# Autodesk Inventor assembly: joint3_frame
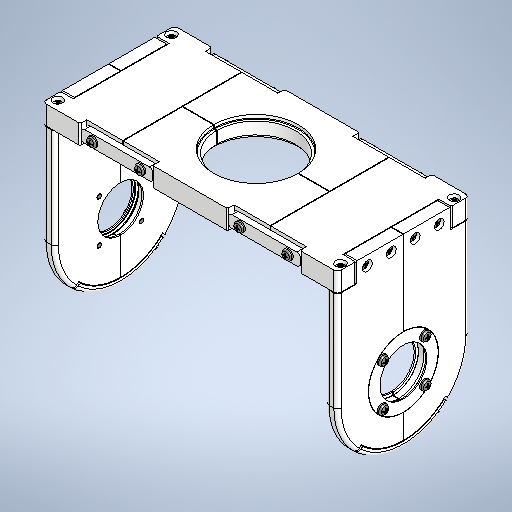
[picture p0: Inventor's stored thumbnail of the model, 512x512]
Saved by Autodesk Inventor 2025.3 (Build 293356030, 356C)
## iProperties
Created: 2025-11-25
Part Number: joint3_frame
Document SubType Name: Assembly
Designer: MSI
Mass: 762.261 g
Surface Area: 1764.87 cm^2
Volume: 601.306 cm^3
Density: 1.26767 g/cm^3
Author: MSI
## Documents named in this file (20)
- C:\Users\MSI\Desktop\Project\3. 로봇팔\Robot Arm Model\joint3\joint3_frame.iam
- C:\Users\MSI\Desktop\Project\3. 로봇팔\Robot Arm Model\joint3\joint3_frame_support1.ipt
- C:\Users\MSI\Desktop\Project\3. 로봇팔\Robot Arm Model\joint3\joint3_frame_support2.ipt
- C:\Users\MSI\Desktop\Project\3. 로봇팔\Robot Arm Model\joint3\joint3_frame1.ipt
- C:\Users\MSI\Desktop\Project\3. 로봇팔\Robot Arm Model\joint3\joint3_frame2.ipt
- C:\Users\MSI\Desktop\Project\3. 로봇팔\Robot Arm Model\joint3\carbon.ipt
- C:\Users\MSI\Desktop\Project\3. 로봇팔\Robot Arm Model\joint3\fixture.ipt
- C:\Users\MSI\Desktop\Project\3. 로봇팔\Robot Arm Model\joint3\joint3_frame_support_fixture.ipt
- C:\Users\MSI\Documents\Inventor\Content Center Files\R2025\ko-KR\KS B 1023  H (2)\KS B 1023 - A  M 4 x 16 - H(1).ipt
- C:\Users\MSI\Desktop\Project\3. 로봇팔\Robot Arm Model\joint3\fixture_MIR2.ipt
- C:\Users\MSI\Desktop\Project\3. 로봇팔\Robot Arm Model\joint3\joint3_frame_cover.ipt
- C:\Users\MSI\Documents\Inventor\Content Center Files\R2025\ko-KR\KS B 1023  H (2)\KS B 1023 - A  M 4 x 10 - H(1).ipt
- C:\Users\MSI\Desktop\Project\3. 로봇팔\Robot Arm Model\joint3\joint3_frame1_MIR.ipt
- C:\Users\MSI\Desktop\Project\3. 로봇팔\Robot Arm Model\joint3\fixture_MIR3.ipt
- C:\Users\MSI\Desktop\Project\3. 로봇팔\Robot Arm Model\joint3\fixture_MIR2_MIR.ipt
- C:\Users\MSI\Desktop\Project\3. 로봇팔\Robot Arm Model\joint3\joint3_frame_support1_MIR.ipt
- C:\Users\MSI\Desktop\Project\3. 로봇팔\Robot Arm Model\joint3\carbon_MIR2.ipt
- C:\Users\MSI\Desktop\Project\3. 로봇팔\Robot Arm Model\joint3\joint3_frame_support2_MIR.ipt
- C:\Users\MSI\Desktop\Project\3. 로봇팔\Robot Arm Model\joint3\joint3_frame_cover_MIR.ipt
- C:\Users\MSI\Desktop\Project\3. 로봇팔\Robot Arm Model\joint3\joint3_frame_support_fixture_MIR.ipt
## Components (64 placed, 19 different names)
1. joint3_frame2:1 — 메이트:1, 메이트:2, 메이트:3, 메이트:4, 메이트:7, 메이트:8, 플러쉬:1, 플러쉬:2, 메이트:9, 메이트:10, 메이트:11, 메이트:12, 메이트:15, 삽입:4, 메이트:56, 삽입:30
2. carbon:1 — 메이트:1, 메이트:2, 메이트:5
3. carbon:2 — 메이트:3, 메이트:4, 메이트:6
4. joint3_frame2:2 — 메이트:5, 메이트:6, 메이트:7, 삽입:8, 삽입:29
5. joint3_frame1:1 — 메이트:13, 메이트:14, 메이트:15, 삽입:3, 삽입:7, 메이트:31, 메이트:32, 메이트:33, 메이트:34, 삽입:14, 삽입:15
6. fixture:1 — 삽입:1, 삽입:2, 삽입:3, 삽입:4
7. KS B 1023 H - 미터 A  M 4 x 16 - H:1 — 삽입:1
8. KS B 1023 H - 미터 A  M 4 x 16 - H:2 — 삽입:2
9. fixture_MIR2:1 — 삽입:5, 삽입:6, 삽입:7, 삽입:8
10. KS B 1023 H - 미터 A  M 4 x 16 - H:3 — 삽입:5
11. KS B 1023 H - 미터 A  M 4 x 16 - H:4 — 삽입:6
12. joint3_frame_support1:1 — 메이트:16, 메이트:17, 메이트:18, 메이트:19, 메이트:20, 메이트:21, 메이트:24, 메이트:25, 삽입:9, 메이트:26, 메이트:28, 메이트:30, 메이트:31, 메이트:33, 삽입:13
13. carbon:11 — 메이트:16, 메이트:17, 메이트:22
14. carbon:12 — 메이트:18, 메이트:19
15. carbon:13 — 메이트:20, 메이트:21, 메이트:23
16. joint3_frame_support2:1 — 메이트:22, 메이트:23, 메이트:24, 메이트:25, 메이트:27, 메이트:29, 메이트:32, 메이트:34
17. joint3_frame_cover:1 — 삽입:9, 메이트:26, 메이트:27, 삽입:10
18. joint3_frame_support_fixture:1 — 메이트:28, 메이트:29, 메이트:30, 삽입:11, 삽입:12
19. KS B 1023 H - 미터 A  M 4 x 16 - H:5 — 삽입:11
20. KS B 1023 H - 미터 A  M 4 x 16 - H:6 — 삽입:12
21. KS B 1023 H - 미터 A  M 4 x 16 - H:8 — 삽입:14
22. KS B 1023 H - 미터 A  M 4 x 16 - H:9 — 삽입:15
23. joint3_frame1_MIR:1 — 메이트:37, 메이트:38, 메이트:39, 메이트:40, 삽입:16, 삽입:19, 삽입:27, 삽입:28, 메이트:54, 메이트:55, 메이트:56
24. fixture_MIR3:1 — 삽입:16, 삽입:17, 삽입:18, 삽입:30
25. KS B 1023 H - 미터 A  M 4 x 16 - H:10 — 삽입:17
26. KS B 1023 H - 미터 A  M 4 x 16 - H:11 — 삽입:18
27. fixture_MIR2_MIR:1 — 삽입:19, 삽입:20, 삽입:21, 삽입:29
28. KS B 1023 H - 미터 A  M 4 x 16 - H:12 — 삽입:20
29. KS B 1023 H - 미터 A  M 4 x 16 - H:13 — 삽입:21
30. joint3_frame_support1_MIR:1 — 메이트:35, 메이트:36, 메이트:38, 메이트:40, 메이트:41, 메이트:43, 삽입:22, 메이트:45, 메이트:47, 메이트:48, 메이트:49, 메이트:50, 메이트:52, 메이트:53, 삽입:26
31. carbon_MIR2:1 — 메이트:46, 메이트:47, 메이트:48
32. carbon_MIR2:2 — 메이트:49, 메이트:50
33. carbon_MIR2:3 — 메이트:51, 메이트:52, 메이트:53
34. joint3_frame_support2_MIR:1 — 메이트:35, 메이트:36, 메이트:37, 메이트:39, 메이트:42, 메이트:44, 메이트:46, 메이트:51
35. joint3_frame_cover_MIR:1 — 삽입:22, 메이트:44, 메이트:45, 삽입:23
36. joint3_frame_support_fixture_MIR:1 — 메이트:41, 메이트:42, 메이트:43, 삽입:24, 삽입:25
37. KS B 1023 H - 미터 A  M 4 x 16 - H:14 — 삽입:24
38. KS B 1023 H - 미터 A  M 4 x 16 - H:15 — 삽입:25
39. KS B 1023 H - 미터 A  M 4 x 16 - H:17 — 삽입:27
40. KS B 1023 H - 미터 A  M 4 x 16 - H:18 — 삽입:28
41. carbon:4 — 메이트:11, 메이트:12, 메이트:54
42. carbon:3 — 메이트:9, 메이트:10, 메이트:13
43. carbon:5
44. carbon:6
45. carbon:7
46. carbon:8
47. carbon:9 — 메이트:55
48. carbon:10 — 메이트:14
49. KS B 1023 H - 미터 A  M 4 x 10 - H:2 — 삽입:23
50. KS B 1023 H - 미터 A  M 4 x 10 - H:1 — 삽입:10
51. KS B 1023 H - 미터 A  M 4 x 10 - H:3
52. KS B 1023 H - 미터 A  M 4 x 10 - H:4
53. KS B 1023 H - 미터 A  M 4 x 10 - H:5
54. KS B 1023 H - 미터 A  M 4 x 10 - H:6
55. KS B 1023 H - 미터 A  M 4 x 10 - H:7
56. KS B 1023 H - 미터 A  M 4 x 10 - H:8
57. KS B 1023 H - 미터 A  M 4 x 16 - H:7 — 삽입:13
58. KS B 1023 H - 미터 A  M 4 x 16 - H:16 — 삽입:26
59. KS B 1023 H - 미터 A  M 4 x 16 - H:19
60. KS B 1023 H - 미터 A  M 4 x 16 - H:20
61. KS B 1023 H - 미터 A  M 4 x 16 - H:21
62. KS B 1023 H - 미터 A  M 4 x 16 - H:22
63. KS B 1023 H - 미터 A  M 4 x 16 - H:23
64. KS B 1023 H - 미터 A  M 4 x 16 - H:24
## Component patterns: (4 elements, first: carbon:4 + carbon:3), (4 elements, first: KS B 1023 H - 미터 A  M 4 x 10 - H:2 + KS B 1023 H - 미터 A  M 4 x 10 - H:1), (4 elements, first: KS B 1023 H - 미터 A  M 4 x 16 - H:7 + KS B 1023 H - 미터 A  M 4 x 16 - H:16)
## Relationships (88: Mate 56, Insert 30, Flush 2)
- 메이트:1 [Mate] (0.25 mm): joint3_frame2:1 ↔ carbon:1
- 메이트:2 [Mate]: joint3_frame2:1 ↔ carbon:1
- 메이트:3 [Mate]: joint3_frame2:1 ↔ carbon:2
- 메이트:4 [Mate]: joint3_frame2:1 ↔ carbon:2
- 메이트:5 [Mate]: carbon:1 ↔ joint3_frame2:2
- 메이트:6 [Mate]: carbon:2 ↔ joint3_frame2:2
- 메이트:7 [Mate] (0.5 mm): joint3_frame2:1 ↔ joint3_frame2:2
- 메이트:8 [Mate]: joint3_frame2:1
- 플러쉬:1 [Flush]: joint3_frame2:1
- 플러쉬:2 [Flush]: joint3_frame2:1
- 메이트:9 [Mate] (0.25 mm): joint3_frame2:1 ↔ carbon:3
- 메이트:10 [Mate]: joint3_frame2:1 ↔ carbon:3
- 메이트:11 [Mate] (0.25 mm): joint3_frame2:1 ↔ carbon:4
- 메이트:12 [Mate]: joint3_frame2:1 ↔ carbon:4
- 메이트:13 [Mate]: joint3_frame1:1 ↔ carbon:3
- 메이트:14 [Mate]: joint3_frame1:1 ↔ carbon:10
- 메이트:15 [Mate] (0.5 mm): joint3_frame2:1 ↔ joint3_frame1:1
- 삽입:1 [Insert]: fixture:1 ↔ KS B 1023 H - 미터 A  M 4 x 16 - H:1
- 삽입:2 [Insert]: fixture:1 ↔ KS B 1023 H - 미터 A  M 4 x 16 - H:2
- 삽입:3 [Insert]: joint3_frame1:1 ↔ fixture:1
- 삽입:4 [Insert]: joint3_frame2:1 ↔ fixture:1
- 삽입:5 [Insert]: fixture_MIR2:1 ↔ KS B 1023 H - 미터 A  M 4 x 16 - H:3
- 삽입:6 [Insert]: fixture_MIR2:1 ↔ KS B 1023 H - 미터 A  M 4 x 16 - H:4
- 삽입:7 [Insert]: joint3_frame1:1 ↔ fixture_MIR2:1
- 삽입:8 [Insert]: joint3_frame2:2 ↔ fixture_MIR2:1
- 메이트:16 [Mate] (0.25 mm): joint3_frame_support1:1 ↔ carbon:11
- 메이트:17 [Mate]: joint3_frame_support1:1 ↔ carbon:11
- 메이트:18 [Mate] (0.25 mm): joint3_frame_support1:1 ↔ carbon:12
- 메이트:19 [Mate]: joint3_frame_support1:1 ↔ carbon:12
- 메이트:20 [Mate] (0.25 mm): joint3_frame_support1:1 ↔ carbon:13
- 메이트:21 [Mate]: joint3_frame_support1:1 ↔ carbon:13
- 메이트:22 [Mate]: carbon:11 ↔ joint3_frame_support2:1
- 메이트:23 [Mate]: carbon:13 ↔ joint3_frame_support2:1
- 메이트:24 [Mate] (0.5 mm): joint3_frame_support1:1 ↔ joint3_frame_support2:1
- 메이트:25 [Mate]: joint3_frame_support1:1 ↔ joint3_frame_support2:1
- 삽입:9 [Insert]: joint3_frame_support1:1 ↔ joint3_frame_cover:1
- 메이트:26 [Mate]: joint3_frame_support1:1 ↔ joint3_frame_cover:1
- 메이트:27 [Mate]: joint3_frame_support2:1 ↔ joint3_frame_cover:1
- 삽입:10 [Insert]: joint3_frame_cover:1 ↔ KS B 1023 H - 미터 A  M 4 x 10 - H:1
- 메이트:28 [Mate]: joint3_frame_support1:1 ↔ joint3_frame_support_fixture:1
- 메이트:29 [Mate]: joint3_frame_support2:1 ↔ joint3_frame_support_fixture:1
- 메이트:30 [Mate]: joint3_frame_support1:1 ↔ joint3_frame_support_fixture:1
- 삽입:11 [Insert]: joint3_frame_support_fixture:1 ↔ KS B 1023 H - 미터 A  M 4 x 16 - H:5
- 삽입:12 [Insert]: joint3_frame_support_fixture:1 ↔ KS B 1023 H - 미터 A  M 4 x 16 - H:6
- 메이트:31 [Mate]: joint3_frame1:1 ↔ joint3_frame_support1:1
- 메이트:32 [Mate]: joint3_frame1:1 ↔ joint3_frame_support2:1
- 메이트:33 [Mate]: joint3_frame1:1 ↔ joint3_frame_support1:1
- 메이트:34 [Mate]: joint3_frame1:1 ↔ joint3_frame_support2:1
- 삽입:13 [Insert]: joint3_frame_support1:1 ↔ KS B 1023 H - 미터 A  M 4 x 16 - H:7
- 삽입:14 [Insert]: joint3_frame1:1 ↔ KS B 1023 H - 미터 A  M 4 x 16 - H:8
- 삽입:15 [Insert]: joint3_frame1:1 ↔ KS B 1023 H - 미터 A  M 4 x 16 - H:9
- 메이트:35 [Mate]: joint3_frame_support1_MIR:1 ↔ joint3_frame_support2_MIR:1
- 메이트:36 [Mate] (0.5 mm): joint3_frame_support1_MIR:1 ↔ joint3_frame_support2_MIR:1
- 메이트:37 [Mate]: joint3_frame1_MIR:1 ↔ joint3_frame_support2_MIR:1
- 메이트:38 [Mate]: joint3_frame1_MIR:1 ↔ joint3_frame_support1_MIR:1
- 메이트:39 [Mate]: joint3_frame1_MIR:1 ↔ joint3_frame_support2_MIR:1
- 메이트:40 [Mate]: joint3_frame1_MIR:1 ↔ joint3_frame_support1_MIR:1
- 삽입:16 [Insert]: joint3_frame1_MIR:1 ↔ fixture_MIR3:1
- 메이트:41 [Mate]: joint3_frame_support1_MIR:1 ↔ joint3_frame_support_fixture_MIR:1
- 메이트:42 [Mate]: joint3_frame_support2_MIR:1 ↔ joint3_frame_support_fixture_MIR:1
- 메이트:43 [Mate]: joint3_frame_support1_MIR:1 ↔ joint3_frame_support_fixture_MIR:1
- 삽입:17 [Insert]: fixture_MIR3:1 ↔ KS B 1023 H - 미터 A  M 4 x 16 - H:10
- 삽입:18 [Insert]: fixture_MIR3:1 ↔ KS B 1023 H - 미터 A  M 4 x 16 - H:11
- 삽입:19 [Insert]: joint3_frame1_MIR:1 ↔ fixture_MIR2_MIR:1
- 삽입:20 [Insert]: fixture_MIR2_MIR:1 ↔ KS B 1023 H - 미터 A  M 4 x 16 - H:12
- 삽입:21 [Insert]: fixture_MIR2_MIR:1 ↔ KS B 1023 H - 미터 A  M 4 x 16 - H:13
- 삽입:22 [Insert]: joint3_frame_support1_MIR:1 ↔ joint3_frame_cover_MIR:1
- 메이트:44 [Mate]: joint3_frame_support2_MIR:1 ↔ joint3_frame_cover_MIR:1
- 메이트:45 [Mate]: joint3_frame_support1_MIR:1 ↔ joint3_frame_cover_MIR:1
- 메이트:46 [Mate]: carbon_MIR2:1 ↔ joint3_frame_support2_MIR:1
- 메이트:47 [Mate]: joint3_frame_support1_MIR:1 ↔ carbon_MIR2:1
- 메이트:48 [Mate] (0.25 mm): joint3_frame_support1_MIR:1 ↔ carbon_MIR2:1
- 메이트:49 [Mate]: joint3_frame_support1_MIR:1 ↔ carbon_MIR2:2
- 메이트:50 [Mate] (0.25 mm): joint3_frame_support1_MIR:1 ↔ carbon_MIR2:2
- 메이트:51 [Mate]: carbon_MIR2:3 ↔ joint3_frame_support2_MIR:1
- 메이트:52 [Mate]: joint3_frame_support1_MIR:1 ↔ carbon_MIR2:3
- 메이트:53 [Mate] (0.25 mm): joint3_frame_support1_MIR:1 ↔ carbon_MIR2:3
- 삽입:23 [Insert]: joint3_frame_cover_MIR:1 ↔ KS B 1023 H - 미터 A  M 4 x 10 - H:2
- 삽입:24 [Insert]: joint3_frame_support_fixture_MIR:1 ↔ KS B 1023 H - 미터 A  M 4 x 16 - H:14
- 삽입:25 [Insert]: joint3_frame_support_fixture_MIR:1 ↔ KS B 1023 H - 미터 A  M 4 x 16 - H:15
- 삽입:26 [Insert]: joint3_frame_support1_MIR:1 ↔ KS B 1023 H - 미터 A  M 4 x 16 - H:16
- 삽입:27 [Insert]: joint3_frame1_MIR:1 ↔ KS B 1023 H - 미터 A  M 4 x 16 - H:17
- 삽입:28 [Insert]: joint3_frame1_MIR:1 ↔ KS B 1023 H - 미터 A  M 4 x 16 - H:18
- 메이트:54 [Mate]: joint3_frame1_MIR:1 ↔ carbon:4
- 메이트:55 [Mate]: joint3_frame1_MIR:1 ↔ carbon:9
- 메이트:56 [Mate] (0.5 mm): joint3_frame2:1 ↔ joint3_frame1_MIR:1
- 삽입:29 [Insert]: joint3_frame2:2 ↔ fixture_MIR2_MIR:1
- 삽입:30 [Insert]: joint3_frame2:1 ↔ fixture_MIR3:1
